# Autodesk Inventor assembly: Zlozenie
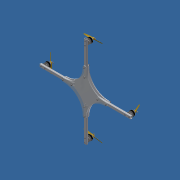
[picture p0: Inventor's stored thumbnail of the model, 180x180]
Saved by Autodesk Inventor 2014 SP1 (Build 180222100, 222)
## iProperties
Created: 2014-08-30
Part Number: Zlozenie
Document SubType Name: Assembly
Designer: Marcin
Author: Marcin
## Documents named in this file (18)
- C:\Users\Marcin\SkyDrive\Dokumenty\Quadrocopter\LabVIEW 3D Model\Zlozenie.iam
- C:\Users\Marcin\SkyDrive\Dokumenty\Quadrocopter\LabVIEW 3D Model\Podstawa.ipt
- C:\Users\Marcin\SkyDrive\Dokumenty\Quadrocopter\LabVIEW 3D Model\Ramie.ipt
- C:\Users\Marcin\SkyDrive\Dokumenty\Quadrocopter\LabVIEW 3D Model\Zlozenie\Design Accelerator\Połączenie gwintowe1.iam
- C:\Users\Marcin\SkyDrive\Dokumenty\Quadrocopter\LabVIEW 3D Model\Zlozenie\Design Accelerator\Połączenie gwintowe2.iam
- C:\Users\Marcin\Documents\Inventor\Content Center Files\R2014\pl-PL\ANSI B18.22 M\ANSI B18.22M - 5 N.ipt
- C:\Users\Marcin\Documents\Inventor\Content Center Files\R2014\pl-PL\ISO 7045(2)\ISO 7045 - M5 x 30 - 4.8 - ZDIN EN ISO.ipt
- C:\Users\Marcin\Documents\Inventor\Content Center Files\R2014\pl-PL\ANSI B18.2.4.2M\ANSI B18.2.4.2M - M5x0.8 - 8.ipt
- C:\Users\Marcin\SkyDrive\Dokumenty\Quadrocopter\LabVIEW 3D Model\Silnik\silnik.iam
- C:\Users\Marcin\SkyDrive\Dokumenty\Quadrocopter\LabVIEW 3D Model\Zlozenie\Design Accelerator\Połączenie gwintowe3.iam
- C:\Users\Marcin\SkyDrive\Dokumenty\Quadrocopter\LabVIEW 3D Model\Zlozenie\Design Accelerator\Połączenie gwintowe4.iam
- C:\Users\Marcin\Documents\Inventor\Content Center Files\R2014\pl-PL\DIN 125-1  A\DIN 125 - A 3.7.ipt
- C:\Users\Marcin\Documents\Inventor\Content Center Files\R2014\pl-PL\JIS B 1101(4)\JIS B 1101 - M3.5 x 20(3).ipt
- C:\Users\Marcin\Documents\Inventor\Content Center Files\R2014\pl-PL\ISO 4035(1)\ISO 4035 - M3.5DIN EN.ipt
- C:\Users\Marcin\SkyDrive\Dokumenty\Quadrocopter\LabVIEW 3D Model\smiglo.ipt
- C:\Users\Marcin\SkyDrive\Dokumenty\Quadrocopter\LabVIEW 3D Model\smiglo-prawe.ipt
- C:\Users\Marcin\SkyDrive\Dokumenty\Quadrocopter\LabVIEW 3D Model\Smiglo-tuleja trzymajaca.ipt
- C:\Users\Marcin\Documents\Inventor\Content Center Files\R2014\pl-PL\ISO 7045(2)\ISO 7045 - M3 x 8 - 4.8 - ZDIN EN ISO.ipt
## Components (87 placed, 14 different names)
1. Podstawa:1 — Zestawiający:1, Zestawiający:2, Zestawiający:3, Równoległy:1, Równoległy:2, Zestawiający:4, Zestawiający:5, Równoległy:3, Zestawiający:6, Zestawiający:7, Zestawiający:8, Równoległy:5, Równoległy:6, Zestawiający:12, Zestawiający:13, Wstaw:9, Wstaw:10, Wstaw:11, Wstaw:12, Wstaw:13, Wstaw:14, Wstaw:15, Wstaw:16, Zestawiający:14, Zestawiający:15
2. Podstawa:2 — Zestawiający:9, Równoległy:5, Równoległy:6, Wstaw:1, Wstaw:2, Wstaw:3, Wstaw:4, Wstaw:5, Wstaw:6, Wstaw:7, Wstaw:8
3. Ramie:1 — Zestawiający:1, Zestawiający:2, Zestawiający:4, Zestawiający:9, Zestawiający:16, Zestawiający:17, Zestawiający:18, Wstaw:35, Wstaw:36
4. silnik:1 [sub-assembly] — Zestawiający:16, Zestawiający:17, Zestawiający:18, Zestawiający:35, Zestawiający:37, Zestawiający:48, Zestawiający:49, Zestawiający:57, Zestawiający:72, Zestawiający:73
5. smiglo:1 — Zestawiający:48, Zestawiający:49, Zestawiający:56
6. Smiglo-tuleja trzymajaca:1 — Zestawiający:56, Zestawiający:57, Zestawiający:64, Zestawiający:65
7. Ramie:2 — Zestawiający:3, Równoległy:1, Równoległy:2, Zestawiający:19, Zestawiający:20, Zestawiający:21, Wstaw:37, Wstaw:38
8. silnik:2 [sub-assembly] — Zestawiający:19, Zestawiający:20, Zestawiający:21, Zestawiający:39, Zestawiający:41, Zestawiający:43, Zestawiający:50, Zestawiający:51
9. smiglo:2 — Zestawiający:50, Zestawiający:51, Zestawiający:60, Zestawiający:61
10. Smiglo-tuleja trzymajaca:3 — Zestawiający:60, Zestawiający:61, Zestawiający:67, Zestawiający:68, Zestawiający:76, Zestawiający:77
11. Ramie:3 — Zestawiający:5, Równoległy:3, Zestawiający:6, Zestawiający:22, Zestawiający:23, Równoległy:7, Wstaw:39, Wstaw:40
12. silnik:3 [sub-assembly] — Zestawiający:22, Zestawiający:23, Równoległy:7, Zestawiający:45, Zestawiający:47, Zestawiający:52, Zestawiający:53, Zestawiający:63
13. smiglo-prawe:2 — Zestawiający:52, Zestawiający:53, Zestawiający:62
14. Smiglo-tuleja trzymajaca:4 — Zestawiający:62, Zestawiający:63, Zestawiający:66, Zestawiający:71, Zestawiający:74, Zestawiający:75
15. Ramie:4 — Zestawiający:7, Zestawiający:8, Równoległy:4, Zestawiający:24, Zestawiający:25, Równoległy:8, Wstaw:33, Wstaw:34
16. silnik:4 [sub-assembly] — Zestawiający:24, Zestawiający:25, Równoległy:8, Zestawiający:26, Zestawiający:27, Zestawiający:28, Zestawiający:29, Zestawiający:31, Zestawiający:33, Zestawiający:54, Zestawiający:55
17. smiglo-prawe:1 — Zestawiający:54, Zestawiający:55, Zestawiający:58, Zestawiający:59
18. Smiglo-tuleja trzymajaca:2 — Zestawiający:58, Zestawiający:59, Zestawiający:69, Zestawiający:70, Zestawiający:78, Zestawiający:79
19. DIN EN ISO 7045 Z M3 x 8 - 4.8 - Z:1 — Zestawiający:64, Zestawiający:73
20. DIN EN ISO 7045 Z M3 x 8 - 4.8 - Z:2 — Zestawiający:65, Zestawiający:72
21. DIN EN ISO 7045 Z M3 x 8 - 4.8 - Z:3 — Zestawiający:66, Zestawiający:74
22. DIN EN ISO 7045 Z M3 x 8 - 4.8 - Z:4 — Zestawiający:67, Zestawiający:76
23. DIN EN ISO 7045 Z M3 x 8 - 4.8 - Z:5 — Zestawiający:68, Zestawiający:77
24. DIN EN ISO 7045 Z M3 x 8 - 4.8 - Z:6 — Zestawiający:69, Zestawiający:79
25. DIN EN ISO 7045 Z M3 x 8 - 4.8 - Z:7 — Zestawiający:70, Zestawiający:78
26. DIN EN ISO 7045 Z M3 x 8 - 4.8 - Z:8 — Zestawiający:71, Zestawiający:75
27. Połączenie gwintowe:1 [sub-assembly] — Zestawiający:14, Zestawiający:15
28. Połączenie gwintowe:2 [sub-assembly] — Zestawiający:12, Zestawiający:13
29. Podkładka okrągła (Metryczny) 5 N:1 — Wstaw:1, Wstaw:17
30. Podkładka okrągła (Metryczny) 5 N:2 — Wstaw:2, Wstaw:19
31. Podkładka okrągła (Metryczny) 5 N:3 — Wstaw:3, Wstaw:24
32. Podkładka okrągła (Metryczny) 5 N:4 — Wstaw:4, Wstaw:22
33. Podkładka okrągła (Metryczny) 5 N:5 — Wstaw:5, Wstaw:21
34. Podkładka okrągła (Metryczny) 5 N:6 — Wstaw:6, Wstaw:23
35. Podkładka okrągła (Metryczny) 5 N:7 — Wstaw:7, Wstaw:20
36. Podkładka okrągła (Metryczny) 5 N:8 — Wstaw:8, Wstaw:18
37. Podkładka okrągła (Metryczny) 5 N:9 — Wstaw:9, Wstaw:26
38. Podkładka okrągła (Metryczny) 5 N:10 — Wstaw:10, Wstaw:27
39. Podkładka okrągła (Metryczny) 5 N:11 — Wstaw:11, Wstaw:32
40. Podkładka okrągła (Metryczny) 5 N:12 — Wstaw:12, Wstaw:30
41. Podkładka okrągła (Metryczny) 5 N:13 — Wstaw:13, Wstaw:29
42. Podkładka okrągła (Metryczny) 5 N:14 — Wstaw:14, Wstaw:31
43. Podkładka okrągła (Metryczny) 5 N:15 — Wstaw:15, Wstaw:28
44. Podkładka okrągła (Metryczny) 5 N:16 — Wstaw:16, Wstaw:25
45. DIN EN ISO 7045 Z M5 x 30 - 4.8 - Z:1 — Wstaw:17
46. DIN EN ISO 7045 Z M5 x 30 - 4.8 - Z:2 — Wstaw:18
47. DIN EN ISO 7045 Z M5 x 30 - 4.8 - Z:3 — Wstaw:19
48. DIN EN ISO 7045 Z M5 x 30 - 4.8 - Z:4 — Wstaw:20
49. DIN EN ISO 7045 Z M5 x 30 - 4.8 - Z:5 — Wstaw:21
50. DIN EN ISO 7045 Z M5 x 30 - 4.8 - Z:6 — Wstaw:22
51. DIN EN ISO 7045 Z M5 x 30 - 4.8 - Z:7 — Wstaw:23
52. DIN EN ISO 7045 Z M5 x 30 - 4.8 - Z:8 — Wstaw:24
53. ANSI B18.2.4.2M M5x0.8:1 — Wstaw:25
54. ANSI B18.2.4.2M M5x0.8:2 — Wstaw:26
55. ANSI B18.2.4.2M M5x0.8:3 — Wstaw:27
56. ANSI B18.2.4.2M M5x0.8:4 — Wstaw:28
57. ANSI B18.2.4.2M M5x0.8:5 — Wstaw:29
58. ANSI B18.2.4.2M M5x0.8:6 — Wstaw:30
59. ANSI B18.2.4.2M M5x0.8:7 — Wstaw:31
60. ANSI B18.2.4.2M M5x0.8:8 — Wstaw:32
61. Połączenie gwintowe:3 [sub-assembly] — Zestawiający:26, Zestawiający:27
62. Połączenie gwintowe:4 [sub-assembly] — Zestawiający:28, Zestawiający:29
63. DIN 125-1 A A 3.7:1 — Wstaw:33, Wstaw:41
64. DIN 125-1 A A 3.7:2 — Wstaw:34, Wstaw:42
65. DIN 125-1 A A 3.7:3 — Wstaw:35, Wstaw:47
66. DIN 125-1 A A 3.7:4 — Wstaw:36, Wstaw:48
67. DIN 125-1 A A 3.7:5 — Wstaw:37, Wstaw:44
68. DIN 125-1 A A 3.7:6 — Wstaw:38, Wstaw:43
69. DIN 125-1 A A 3.7:7 — Wstaw:39, Wstaw:45
70. DIN 125-1 A A 3.7:8 — Wstaw:40, Wstaw:46
71. JIS B 1101 - zgodne z ISO 1580 - Metryczny M3.5 x 20:1 — Wstaw:41, Zestawiający:30
72. JIS B 1101 - zgodne z ISO 1580 - Metryczny M3.5 x 20:2 — Wstaw:42, Zestawiający:32
73. DIN EN 24035 M3.5:1 — Zestawiający:30, Zestawiający:31
74. DIN EN 24035 M3.5:2 — Zestawiający:32, Zestawiający:33
75. JIS B 1101 - zgodne z ISO 1580 - Metryczny M3.5 x 20:3 — Wstaw:43, Zestawiający:38, Zestawiający:42
76. JIS B 1101 - zgodne z ISO 1580 - Metryczny M3.5 x 20:4 — Wstaw:44, Zestawiający:40
77. JIS B 1101 - zgodne z ISO 1580 - Metryczny M3.5 x 20:5 — Wstaw:45, Zestawiający:44
78. JIS B 1101 - zgodne z ISO 1580 - Metryczny M3.5 x 20:6 — Wstaw:46, Zestawiający:46
79. JIS B 1101 - zgodne z ISO 1580 - Metryczny M3.5 x 20:7 — Wstaw:47, Zestawiający:34
80. JIS B 1101 - zgodne z ISO 1580 - Metryczny M3.5 x 20:8 — Wstaw:48, Zestawiający:36
81. DIN EN 24035 M3.5:3 — Zestawiający:34, Zestawiający:35
82. DIN EN 24035 M3.5:4 — Zestawiający:36, Zestawiający:37
83. DIN EN 24035 M3.5:5 — Zestawiający:38, Zestawiający:39
84. DIN EN 24035 M3.5:6 — Zestawiający:40, Zestawiający:41
85. DIN EN 24035 M3.5:7 — Zestawiający:42, Zestawiający:43
86. DIN EN 24035 M3.5:8 — Zestawiający:44, Zestawiający:45
87. DIN EN 24035 M3.5:9 — Zestawiający:46, Zestawiający:47
## Relationships (133: Mate 77, Insert 48, Flush 8)
- Zestawiający:1 [Mate]: Podstawa:1 ↔ Ramie:1
- Zestawiający:2 [Mate] (-70 mm): Podstawa:1 ↔ Ramie:1
- Zestawiający:3 [Mate]: Podstawa:1 ↔ Ramie:2
- Równoległy:1 [Flush] (70 mm): Podstawa:1 ↔ Ramie:2
- Równoległy:2 [Flush] (0.032 mm): Podstawa:1 ↔ Ramie:2
- Zestawiający:4 [Mate] (0.032 mm): Podstawa:1 ↔ Ramie:1
- Zestawiający:5 [Mate]: Podstawa:1 ↔ Ramie:3
- Równoległy:3 [Flush] (-70 mm): Podstawa:1 ↔ Ramie:3
- Zestawiający:6 [Mate] (0.032 mm): Podstawa:1 ↔ Ramie:3
- Zestawiający:7 [Mate]: Podstawa:1 ↔ Ramie:4
- Zestawiający:8 [Mate] (-70 mm): Podstawa:1 ↔ Ramie:4
- Równoległy:4 [Flush]: Ramie:4
- Zestawiający:9 [Mate]: Podstawa:2 ↔ Ramie:1
- Równoległy:5 [Flush]: Podstawa:1 ↔ Podstawa:2
- Równoległy:6 [Flush]: Podstawa:1 ↔ Podstawa:2
- Zestawiający:12 [Mate]: Podstawa:1 ↔ Połączenie gwintowe:2
- Zestawiający:13 [Mate]: Podstawa:1 ↔ Połączenie gwintowe:2
- Wstaw:1 [Insert]: Podstawa:2 ↔ Podkładka okrągła (Metryczny) 5 N:1
- Wstaw:2 [Insert]: Podstawa:2 ↔ Podkładka okrągła (Metryczny) 5 N:2
- Wstaw:3 [Insert]: Podstawa:2 ↔ Podkładka okrągła (Metryczny) 5 N:3
- Wstaw:4 [Insert]: Podstawa:2 ↔ Podkładka okrągła (Metryczny) 5 N:4
- Wstaw:5 [Insert]: Podstawa:2 ↔ Podkładka okrągła (Metryczny) 5 N:5
- Wstaw:6 [Insert]: Podstawa:2 ↔ Podkładka okrągła (Metryczny) 5 N:6
- Wstaw:7 [Insert]: Podstawa:2 ↔ Podkładka okrągła (Metryczny) 5 N:7
- Wstaw:8 [Insert]: Podstawa:2 ↔ Podkładka okrągła (Metryczny) 5 N:8
- Wstaw:9 [Insert]: Podstawa:1 ↔ Podkładka okrągła (Metryczny) 5 N:9
- Wstaw:10 [Insert]: Podstawa:1 ↔ Podkładka okrągła (Metryczny) 5 N:10
- Wstaw:11 [Insert]: Podstawa:1 ↔ Podkładka okrągła (Metryczny) 5 N:11
- Wstaw:12 [Insert]: Podstawa:1 ↔ Podkładka okrągła (Metryczny) 5 N:12
- Wstaw:13 [Insert]: Podstawa:1 ↔ Podkładka okrągła (Metryczny) 5 N:13
- Wstaw:14 [Insert]: Podstawa:1 ↔ Podkładka okrągła (Metryczny) 5 N:14
- Wstaw:15 [Insert]: Podstawa:1 ↔ Podkładka okrągła (Metryczny) 5 N:15
- Wstaw:16 [Insert]: Podstawa:1 ↔ Podkładka okrągła (Metryczny) 5 N:16
- Wstaw:17 [Insert]: Podkładka okrągła (Metryczny) 5 N:1 ↔ DIN EN ISO 7045 Z M5 x 30 - 4.8 - Z:1
- Wstaw:18 [Insert]: Podkładka okrągła (Metryczny) 5 N:8 ↔ DIN EN ISO 7045 Z M5 x 30 - 4.8 - Z:2
- Wstaw:19 [Insert]: Podkładka okrągła (Metryczny) 5 N:2 ↔ DIN EN ISO 7045 Z M5 x 30 - 4.8 - Z:3
- Wstaw:20 [Insert]: Podkładka okrągła (Metryczny) 5 N:7 ↔ DIN EN ISO 7045 Z M5 x 30 - 4.8 - Z:4
- Wstaw:21 [Insert]: Podkładka okrągła (Metryczny) 5 N:5 ↔ DIN EN ISO 7045 Z M5 x 30 - 4.8 - Z:5
- Wstaw:22 [Insert]: Podkładka okrągła (Metryczny) 5 N:4 ↔ DIN EN ISO 7045 Z M5 x 30 - 4.8 - Z:6
- Wstaw:23 [Insert]: Podkładka okrągła (Metryczny) 5 N:6 ↔ DIN EN ISO 7045 Z M5 x 30 - 4.8 - Z:7
- Wstaw:24 [Insert]: Podkładka okrągła (Metryczny) 5 N:3 ↔ DIN EN ISO 7045 Z M5 x 30 - 4.8 - Z:8
- Wstaw:25 [Insert]: Podkładka okrągła (Metryczny) 5 N:16 ↔ ANSI B18.2.4.2M M5x0.8:1
- Wstaw:26 [Insert]: Podkładka okrągła (Metryczny) 5 N:9 ↔ ANSI B18.2.4.2M M5x0.8:2
- Wstaw:27 [Insert]: Podkładka okrągła (Metryczny) 5 N:10 ↔ ANSI B18.2.4.2M M5x0.8:3
- Wstaw:28 [Insert]: Podkładka okrągła (Metryczny) 5 N:15 ↔ ANSI B18.2.4.2M M5x0.8:4
- Wstaw:29 [Insert]: Podkładka okrągła (Metryczny) 5 N:13 ↔ ANSI B18.2.4.2M M5x0.8:5
- Wstaw:30 [Insert]: Podkładka okrągła (Metryczny) 5 N:12 ↔ ANSI B18.2.4.2M M5x0.8:6
- Wstaw:31 [Insert]: Podkładka okrągła (Metryczny) 5 N:14 ↔ ANSI B18.2.4.2M M5x0.8:7
- Wstaw:32 [Insert]: Podkładka okrągła (Metryczny) 5 N:11 ↔ ANSI B18.2.4.2M M5x0.8:8
- Zestawiający:14 [Mate]: Podstawa:1 ↔ Połączenie gwintowe:1
- Zestawiający:15 [Mate]: Podstawa:1 ↔ Połączenie gwintowe:1
- Zestawiający:16 [Mate]: Ramie:1 ↔ silnik:1
- Zestawiający:17 [Mate]: Ramie:1 ↔ silnik:1
- Zestawiający:18 [Mate] (-20 mm): Ramie:1 ↔ silnik:1
- Zestawiający:19 [Mate]: Ramie:2 ↔ silnik:2
- Zestawiający:20 [Mate]: Ramie:2 ↔ silnik:2
- Zestawiający:21 [Mate] (-20 mm): Ramie:2 ↔ silnik:2
- Zestawiający:22 [Mate]: Ramie:3 ↔ silnik:3
- Zestawiający:23 [Mate]: Ramie:3 ↔ silnik:3
- Równoległy:7 [Flush] (20 mm): Ramie:3 ↔ silnik:3
- Zestawiający:24 [Mate]: Ramie:4 ↔ silnik:4
- Zestawiający:25 [Mate]: Ramie:4 ↔ silnik:4
- Równoległy:8 [Flush] (20 mm): Ramie:4 ↔ silnik:4
- Zestawiający:26 [Mate]: silnik:4 ↔ Połączenie gwintowe:3
- Zestawiający:27 [Mate]: silnik:4 ↔ Połączenie gwintowe:3
- Zestawiający:28 [Mate]: silnik:4 ↔ Połączenie gwintowe:4
- Zestawiający:29 [Mate]: silnik:4 ↔ Połączenie gwintowe:4
- Wstaw:33 [Insert]: Ramie:4 ↔ DIN 125-1 A A 3.7:1
- Wstaw:34 [Insert]: Ramie:4 ↔ DIN 125-1 A A 3.7:2
- Wstaw:35 [Insert]: Ramie:1 ↔ DIN 125-1 A A 3.7:3
- Wstaw:36 [Insert]: Ramie:1 ↔ DIN 125-1 A A 3.7:4
- Wstaw:37 [Insert]: Ramie:2 ↔ DIN 125-1 A A 3.7:5
- Wstaw:38 [Insert]: Ramie:2 ↔ DIN 125-1 A A 3.7:6
- Wstaw:39 [Insert]: Ramie:3 ↔ DIN 125-1 A A 3.7:7
- Wstaw:40 [Insert]: Ramie:3 ↔ DIN 125-1 A A 3.7:8
- Wstaw:41 [Insert]: DIN 125-1 A A 3.7:1 ↔ JIS B 1101 - zgodne z ISO 1580 - Metryczny M3.5 x 20:1
- Wstaw:42 [Insert]: DIN 125-1 A A 3.7:2 ↔ JIS B 1101 - zgodne z ISO 1580 - Metryczny M3.5 x 20:2
- Zestawiający:30 [Mate]: JIS B 1101 - zgodne z ISO 1580 - Metryczny M3.5 x 20:1 ↔ DIN EN 24035 M3.5:1
- Zestawiający:31 [Mate]: silnik:4 ↔ DIN EN 24035 M3.5:1
- Zestawiający:32 [Mate]: JIS B 1101 - zgodne z ISO 1580 - Metryczny M3.5 x 20:2 ↔ DIN EN 24035 M3.5:2
- Zestawiający:33 [Mate]: silnik:4 ↔ DIN EN 24035 M3.5:2
- Wstaw:43 [Insert]: DIN 125-1 A A 3.7:6 ↔ JIS B 1101 - zgodne z ISO 1580 - Metryczny M3.5 x 20:3
- Wstaw:44 [Insert]: DIN 125-1 A A 3.7:5 ↔ JIS B 1101 - zgodne z ISO 1580 - Metryczny M3.5 x 20:4
- Wstaw:45 [Insert]: DIN 125-1 A A 3.7:7 ↔ JIS B 1101 - zgodne z ISO 1580 - Metryczny M3.5 x 20:5
- Wstaw:46 [Insert]: DIN 125-1 A A 3.7:8 ↔ JIS B 1101 - zgodne z ISO 1580 - Metryczny M3.5 x 20:6
- Wstaw:47 [Insert]: DIN 125-1 A A 3.7:3 ↔ JIS B 1101 - zgodne z ISO 1580 - Metryczny M3.5 x 20:7
- Wstaw:48 [Insert]: DIN 125-1 A A 3.7:4 ↔ JIS B 1101 - zgodne z ISO 1580 - Metryczny M3.5 x 20:8
- Zestawiający:34 [Mate]: JIS B 1101 - zgodne z ISO 1580 - Metryczny M3.5 x 20:7 ↔ DIN EN 24035 M3.5:3
- Zestawiający:35 [Mate]: silnik:1 ↔ DIN EN 24035 M3.5:3
- Zestawiający:36 [Mate]: JIS B 1101 - zgodne z ISO 1580 - Metryczny M3.5 x 20:8 ↔ DIN EN 24035 M3.5:4
- Zestawiający:37 [Mate]: silnik:1 ↔ DIN EN 24035 M3.5:4
- Zestawiający:38 [Mate]: JIS B 1101 - zgodne z ISO 1580 - Metryczny M3.5 x 20:3 ↔ DIN EN 24035 M3.5:5
- Zestawiający:39 [Mate]: silnik:2 ↔ DIN EN 24035 M3.5:5
- Zestawiający:40 [Mate]: JIS B 1101 - zgodne z ISO 1580 - Metryczny M3.5 x 20:4 ↔ DIN EN 24035 M3.5:6
- Zestawiający:41 [Mate]: silnik:2 ↔ DIN EN 24035 M3.5:6
- Zestawiający:42 [Mate]: JIS B 1101 - zgodne z ISO 1580 - Metryczny M3.5 x 20:3 ↔ DIN EN 24035 M3.5:7
- Zestawiający:43 [Mate]: silnik:2 ↔ DIN EN 24035 M3.5:7
- Zestawiający:44 [Mate]: JIS B 1101 - zgodne z ISO 1580 - Metryczny M3.5 x 20:5 ↔ DIN EN 24035 M3.5:8
- Zestawiający:45 [Mate]: silnik:3 ↔ DIN EN 24035 M3.5:8
- Zestawiający:46 [Mate]: JIS B 1101 - zgodne z ISO 1580 - Metryczny M3.5 x 20:6 ↔ DIN EN 24035 M3.5:9
- Zestawiający:47 [Mate]: silnik:3 ↔ DIN EN 24035 M3.5:9
- Zestawiający:48 [Mate]: silnik:1 ↔ smiglo:1
- Zestawiający:49 [Mate]: silnik:1 ↔ smiglo:1
- Zestawiający:50 [Mate]: silnik:2 ↔ smiglo:2
- Zestawiający:51 [Mate]: silnik:2 ↔ smiglo:2
- Zestawiający:52 [Mate]: silnik:3 ↔ smiglo-prawe:2
- Zestawiający:53 [Mate]: silnik:3 ↔ smiglo-prawe:2
- Zestawiający:54 [Mate]: silnik:4 ↔ smiglo-prawe:1
- Zestawiający:55 [Mate]: silnik:4 ↔ smiglo-prawe:1
- Zestawiający:56 [Mate]: smiglo:1 ↔ Smiglo-tuleja trzymajaca:1
- Zestawiający:57 [Mate]: silnik:1 ↔ Smiglo-tuleja trzymajaca:1
- Zestawiający:58 [Mate]: smiglo-prawe:1 ↔ Smiglo-tuleja trzymajaca:2
- Zestawiający:59 [Mate]: smiglo-prawe:1 ↔ Smiglo-tuleja trzymajaca:2
- Zestawiający:60 [Mate]: smiglo:2 ↔ Smiglo-tuleja trzymajaca:3
- Zestawiający:61 [Mate]: smiglo:2 ↔ Smiglo-tuleja trzymajaca:3
- Zestawiający:62 [Mate]: smiglo-prawe:2 ↔ Smiglo-tuleja trzymajaca:4
- Zestawiający:63 [Mate]: silnik:3 ↔ Smiglo-tuleja trzymajaca:4
- Zestawiający:64 [Mate]: Smiglo-tuleja trzymajaca:1 ↔ DIN EN ISO 7045 Z M3 x 8 - 4.8 - Z:1
- Zestawiający:65 [Mate]: Smiglo-tuleja trzymajaca:1 ↔ DIN EN ISO 7045 Z M3 x 8 - 4.8 - Z:2
- Zestawiający:66 [Mate]: Smiglo-tuleja trzymajaca:4 ↔ DIN EN ISO 7045 Z M3 x 8 - 4.8 - Z:3
- Zestawiający:67 [Mate]: Smiglo-tuleja trzymajaca:3 ↔ DIN EN ISO 7045 Z M3 x 8 - 4.8 - Z:4
- Zestawiający:68 [Mate]: Smiglo-tuleja trzymajaca:3 ↔ DIN EN ISO 7045 Z M3 x 8 - 4.8 - Z:5
- Zestawiający:69 [Mate]: Smiglo-tuleja trzymajaca:2 ↔ DIN EN ISO 7045 Z M3 x 8 - 4.8 - Z:6
- Zestawiający:70 [Mate]: Smiglo-tuleja trzymajaca:2 ↔ DIN EN ISO 7045 Z M3 x 8 - 4.8 - Z:7
- Zestawiający:71 [Mate]: Smiglo-tuleja trzymajaca:4 ↔ DIN EN ISO 7045 Z M3 x 8 - 4.8 - Z:8
- Zestawiający:72 [Mate] (1.5 mm): silnik:1 ↔ DIN EN ISO 7045 Z M3 x 8 - 4.8 - Z:2
- Zestawiający:73 [Mate] (1.5 mm): silnik:1 ↔ DIN EN ISO 7045 Z M3 x 8 - 4.8 - Z:1
- Zestawiający:74 [Mate] (1.5 mm): Smiglo-tuleja trzymajaca:4 ↔ DIN EN ISO 7045 Z M3 x 8 - 4.8 - Z:3
- Zestawiający:75 [Mate] (1.5 mm): Smiglo-tuleja trzymajaca:4 ↔ DIN EN ISO 7045 Z M3 x 8 - 4.8 - Z:8
- Zestawiający:76 [Mate] (1.5 mm): Smiglo-tuleja trzymajaca:3 ↔ DIN EN ISO 7045 Z M3 x 8 - 4.8 - Z:4
- Zestawiający:77 [Mate] (1.5 mm): Smiglo-tuleja trzymajaca:3 ↔ DIN EN ISO 7045 Z M3 x 8 - 4.8 - Z:5
- Zestawiający:78 [Mate] (1.5 mm): Smiglo-tuleja trzymajaca:2 ↔ DIN EN ISO 7045 Z M3 x 8 - 4.8 - Z:7
- Zestawiający:79 [Mate] (1.5 mm): Smiglo-tuleja trzymajaca:2 ↔ DIN EN ISO 7045 Z M3 x 8 - 4.8 - Z:6
